# Autodesk Inventor assembly: Car Assembly - Solo_MIR
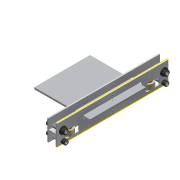
[picture p0: Inventor's stored thumbnail of the model, 180x180]
Saved by Autodesk Inventor 2015 (Build 190159000, 159)
## iProperties
Created: 2014-07-18
Part Number: Car Assembly - Solo_MIR
Document SubType Name: Assembly
Designer: Peter
Author: Owner
## Documents named in this file (9)
- T:\FILES\Inventor 2015 Projects\Elevator Version 2\Frc Chassis 2014\Car Assembly - Solo_MIR.iam
- T:\FILES\Inventor 2015 Projects\Elevator Version 2\Frc Chassis 2014\car frame_MIR.ipt
- T:\FILES\Inventor 2015 Projects\Elevator Version 2\Frc Chassis 2014\#8 .5 Hex Standoff_MIR.ipt
- T:\FILES\Inventor 2015 Projects\Elevator Version 2\Frc Chassis 2014\.25 #8 .3125 Spacer_MIR.ipt
- T:\FILES\Inventor 2015 Projects\Elevator Version 2\Frc Chassis 2014\Flange Sleve Bearing .25.375 _MIR.ipt
- T:\FILES\Inventor 2015 Projects\Elevator Version 2\Frc Chassis 2014\Sleeve Bearing .25 .3125 _MIR.ipt
- T:\FILES\Inventor 2015 Projects\Elevator Version 2\Frc Chassis 2014\.375 .75 .375 Nylon Spacer_MIR.ipt
- T:\FILES\Inventor 2015 Projects\Elevator Version 2\Frc Chassis 2014\.25 #8 .5625 Spacer_MIR.ipt
- T:\FILES\Inventor 2015 Projects\Elevator Version 2\Frc Chassis 2014\Inter-rail plate_MIR.ipt
## Components (30 placed, 8 different names)
1. car frame_MIR:1 — Mate:17, Mate:16, Mate:2, Mate:1, Mate:31, Mate:30, Mate:33, Mate:32, Mate:48, Mate:46, Mate:35, Mate:34, Mate:14, Mate:13, Mate:23, Mate:22, Mate:9, Mate:8, Mate:4, Mate:3, Mate:41, Mate:39, Mate:40, Mate:38, Mate:47, Mate:24, Mate:44, Mate:18, Mate:42, Mate:36, Mate:82, Mate:75, Mate:81, Mate:74, Mate:80, Mate:79, Mate:78
2. #8 .5 Hex Standoff_MIR:1 — Mate:17, Mate:16
3. #8 .5 Hex Standoff_MIR:2 — Mate:2, Mate:1
4. #8 .5 Hex Standoff_MIR:3 — Mate:31, Mate:30
5. #8 .5 Hex Standoff_MIR:4 — Mate:33, Mate:32
6. .25 #8 .3125 Spacer_MIR:1 — Mate:48, Mate:46, Mate:49
7. .25 #8 .3125 Spacer_MIR:2 — Mate:35, Mate:34, Mate:37
8. .25 #8 .3125 Spacer_MIR:3 — Mate:14, Mate:13, Mate:19
9. .25 #8 .3125 Spacer_MIR:4 — Mate:23, Mate:22, Mate:25
10. .25 #8 .3125 Spacer_MIR:5 — Mate:9, Mate:8, Mate:10, Flush:2
11. .25 #8 .3125 Spacer_MIR:6 — Mate:4, Mate:3, Flush:1, Mate:5
12. .25 #8 .3125 Spacer_MIR:7 — Mate:41, Mate:39, Mate:45
13. .25 #8 .3125 Spacer_MIR:8 — Mate:40, Mate:38, Mate:43
14. Flange Sleve Bearing .25.375 _MIR:1 — Mate:47, Mate:49
15. Flange Sleve Bearing .25.375 _MIR:2 — Mate:24, Mate:25
16. Flange Sleve Bearing .25.375 _MIR:3 — Mate:45, Mate:44
17. Flange Sleve Bearing .25.375 _MIR:4 — Mate:18, Mate:19
18. Sleeve Bearing .25 .3125 _MIR:1 — Mate:43, Mate:42
19. Sleeve Bearing .25 .3125 _MIR:2 — Mate:37, Mate:36
20. Sleeve Bearing .25 .3125 _MIR:3 — Mate:10, Flush:2
21. Sleeve Bearing .25 .3125 _MIR:4 — Flush:1, Mate:5
22. .375 .75 .375 Nylon Spacer_MIR:1 — Mate:64, Mate:63, Mate:60, Mate:58
23. .375 .75 .375 Nylon Spacer_MIR:2 — Mate:65, Mate:62, Mate:61, Mate:59
24. Flange Sleve Bearing .25.375 _MIR:5 — Mate:64, Mate:63, Mate:66
25. Flange Sleve Bearing .25.375 _MIR:6 — Mate:65, Mate:62, Mate:67
26. Flange Sleve Bearing .25.375 _MIR:7 — Mate:60, Mate:58, Mate:69
27. Flange Sleve Bearing .25.375 _MIR:8 — Mate:61, Mate:59, Mate:68
28. .25 #8 .5625 Spacer_MIR:1 — Mate:82, Mate:75, Mate:69, Mate:66
29. .25 #8 .5625 Spacer_MIR:2 — Mate:81, Mate:74, Mate:68, Mate:67
30. Inter-rail plate_MIR:1 — Mate:80, Mate:79, Mate:78
## Relationships (59: Mate 57, Flush 2)
- Mate:17: car frame_MIR:1 ↔ #8 .5 Hex Standoff_MIR:1
- Mate:16: car frame_MIR:1 ↔ #8 .5 Hex Standoff_MIR:1
- Mate:2: car frame_MIR:1 ↔ #8 .5 Hex Standoff_MIR:2
- Mate:1: car frame_MIR:1 ↔ #8 .5 Hex Standoff_MIR:2
- Mate:31: car frame_MIR:1 ↔ #8 .5 Hex Standoff_MIR:3
- Mate:30: car frame_MIR:1 ↔ #8 .5 Hex Standoff_MIR:3
- Mate:33: car frame_MIR:1 ↔ #8 .5 Hex Standoff_MIR:4
- Mate:32: car frame_MIR:1 ↔ #8 .5 Hex Standoff_MIR:4
- Mate:48: car frame_MIR:1 ↔ .25 #8 .3125 Spacer_MIR:1
- Mate:46: car frame_MIR:1 ↔ .25 #8 .3125 Spacer_MIR:1
- Mate:35: car frame_MIR:1 ↔ .25 #8 .3125 Spacer_MIR:2
- Mate:34: car frame_MIR:1 ↔ .25 #8 .3125 Spacer_MIR:2
- Mate:14: car frame_MIR:1 ↔ .25 #8 .3125 Spacer_MIR:3
- Mate:13: car frame_MIR:1 ↔ .25 #8 .3125 Spacer_MIR:3
- Mate:23: car frame_MIR:1 ↔ .25 #8 .3125 Spacer_MIR:4
- Mate:22: car frame_MIR:1 ↔ .25 #8 .3125 Spacer_MIR:4
- Mate:9: car frame_MIR:1 ↔ .25 #8 .3125 Spacer_MIR:5
- Mate:8: car frame_MIR:1 ↔ .25 #8 .3125 Spacer_MIR:5
- Mate:4: car frame_MIR:1 ↔ .25 #8 .3125 Spacer_MIR:6
- Mate:3: car frame_MIR:1 ↔ .25 #8 .3125 Spacer_MIR:6
- Mate:41: car frame_MIR:1 ↔ .25 #8 .3125 Spacer_MIR:7
- Mate:39: car frame_MIR:1 ↔ .25 #8 .3125 Spacer_MIR:7
- Mate:40: car frame_MIR:1 ↔ .25 #8 .3125 Spacer_MIR:8
- Mate:38: car frame_MIR:1 ↔ .25 #8 .3125 Spacer_MIR:8
- Mate:47 (0.635 mm): car frame_MIR:1 ↔ Flange Sleve Bearing .25.375 _MIR:1
- Mate:49: .25 #8 .3125 Spacer_MIR:1 ↔ Flange Sleve Bearing .25.375 _MIR:1
- Mate:24 (0.635 mm): car frame_MIR:1 ↔ Flange Sleve Bearing .25.375 _MIR:2
- Mate:25: .25 #8 .3125 Spacer_MIR:4 ↔ Flange Sleve Bearing .25.375 _MIR:2
- Mate:45: .25 #8 .3125 Spacer_MIR:7 ↔ Flange Sleve Bearing .25.375 _MIR:3
- Mate:44 (0.635 mm): car frame_MIR:1 ↔ Flange Sleve Bearing .25.375 _MIR:3
- Mate:18 (0.635 mm): car frame_MIR:1 ↔ Flange Sleve Bearing .25.375 _MIR:4
- Mate:19: .25 #8 .3125 Spacer_MIR:3 ↔ Flange Sleve Bearing .25.375 _MIR:4
- Mate:43: .25 #8 .3125 Spacer_MIR:8 ↔ Sleeve Bearing .25 .3125 _MIR:1
- Mate:42 (0.635 mm): car frame_MIR:1 ↔ Sleeve Bearing .25 .3125 _MIR:1
- Mate:37: .25 #8 .3125 Spacer_MIR:2 ↔ Sleeve Bearing .25 .3125 _MIR:2
- Mate:36 (-0.635 mm): car frame_MIR:1 ↔ Sleeve Bearing .25 .3125 _MIR:2
- Mate:10: .25 #8 .3125 Spacer_MIR:5 ↔ Sleeve Bearing .25 .3125 _MIR:3
- Flush:2: .25 #8 .3125 Spacer_MIR:5 ↔ Sleeve Bearing .25 .3125 _MIR:3
- Flush:1: .25 #8 .3125 Spacer_MIR:6 ↔ Sleeve Bearing .25 .3125 _MIR:4
- Mate:5: .25 #8 .3125 Spacer_MIR:6 ↔ Sleeve Bearing .25 .3125 _MIR:4
- Mate:64: .375 .75 .375 Nylon Spacer_MIR:1 ↔ Flange Sleve Bearing .25.375 _MIR:5
- Mate:63: .375 .75 .375 Nylon Spacer_MIR:1 ↔ Flange Sleve Bearing .25.375 _MIR:5
- Mate:65: .375 .75 .375 Nylon Spacer_MIR:2 ↔ Flange Sleve Bearing .25.375 _MIR:6
- Mate:62: .375 .75 .375 Nylon Spacer_MIR:2 ↔ Flange Sleve Bearing .25.375 _MIR:6
- Mate:60: .375 .75 .375 Nylon Spacer_MIR:1 ↔ Flange Sleve Bearing .25.375 _MIR:7
- Mate:58: .375 .75 .375 Nylon Spacer_MIR:1 ↔ Flange Sleve Bearing .25.375 _MIR:7
- Mate:61: .375 .75 .375 Nylon Spacer_MIR:2 ↔ Flange Sleve Bearing .25.375 _MIR:8
- Mate:59: .375 .75 .375 Nylon Spacer_MIR:2 ↔ Flange Sleve Bearing .25.375 _MIR:8
- Mate:82: car frame_MIR:1 ↔ .25 #8 .5625 Spacer_MIR:1
- Mate:75: car frame_MIR:1 ↔ .25 #8 .5625 Spacer_MIR:1
- Mate:69 (0.635 mm): Flange Sleve Bearing .25.375 _MIR:7 ↔ .25 #8 .5625 Spacer_MIR:1
- Mate:66: Flange Sleve Bearing .25.375 _MIR:5 ↔ .25 #8 .5625 Spacer_MIR:1
- Mate:81: car frame_MIR:1 ↔ .25 #8 .5625 Spacer_MIR:2
- Mate:74: car frame_MIR:1 ↔ .25 #8 .5625 Spacer_MIR:2
- Mate:68 (0.635 mm): Flange Sleve Bearing .25.375 _MIR:8 ↔ .25 #8 .5625 Spacer_MIR:2
- Mate:67: Flange Sleve Bearing .25.375 _MIR:6 ↔ .25 #8 .5625 Spacer_MIR:2
- Mate:80 (9.525 mm): car frame_MIR:1 ↔ Inter-rail plate_MIR:1
- Mate:79: car frame_MIR:1 ↔ Inter-rail plate_MIR:1
- Mate:78: car frame_MIR:1 ↔ Inter-rail plate_MIR:1
